# Autodesk Inventor assembly: Chewbacca
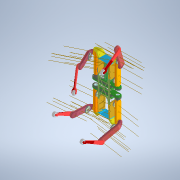
[picture p0: Inventor's stored thumbnail of the model, 180x180]
Saved by Autodesk Inventor 2022.2 (Build 262287000, 287)
## iProperties
Created: 2022-01-14
Part Number: Chewbacca
Document SubType Name: Assembly
Designer: Jochen
Author: Jochen
## Documents named in this file (5)
- D:\Projects\Chewbacca\CAD\Chewbacca.iam
- D:\Projects\Chewbacca\CAD\BodyStructure.iam
- D:\Projects\Chewbacca\CAD\Leg Long.iam
- D:\Projects\Chewbacca\CAD\Leg Short.iam
- D:\Projects\Chewbacca\CAD\Common\odrive\ODrive Pack.iam
## Components (6 placed, 4 different names)
1. BodyStructure:1 [sub-assembly] — Mate:1, Mate:5, Mate:7, Mate:8, Mate:9, Mate:10, Mate:11, Mate:12, Mate:18, Mate:19
2. Leg Long:1 [sub-assembly] — Mate:5, Mate:8
3. Leg Short:1 [sub-assembly] — Mate:1, Mate:7
4. Leg Long:2 [sub-assembly] — Mate:9, Mate:10
5. Leg Short:2 [sub-assembly] — Mate:11, Mate:12
6. ODrive Pack:1 [sub-assembly] — Mate:18, Mate:19
## Relationships (10: Mate 10)
- Mate:1: BodyStructure:1 ↔ Leg Short:1
- Mate:5: BodyStructure:1 ↔ Leg Long:1
- Mate:7: BodyStructure:1 ↔ Leg Short:1
- Mate:8: BodyStructure:1 ↔ Leg Long:1
- Mate:9: BodyStructure:1 ↔ Leg Long:2
- Mate:10: BodyStructure:1 ↔ Leg Long:2
- Mate:11: BodyStructure:1 ↔ Leg Short:2
- Mate:12: BodyStructure:1 ↔ Leg Short:2
- Mate:18: BodyStructure:1 ↔ ODrive Pack:1
- Mate:19: BodyStructure:1 ↔ ODrive Pack:1
